# Autodesk Inventor assembly: Złożenie
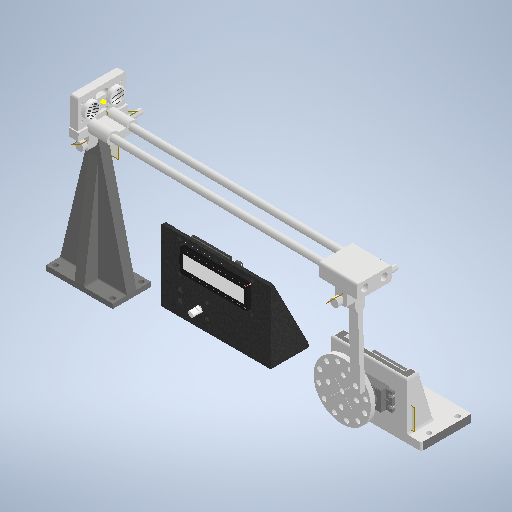
[picture p0: Inventor's stored thumbnail of the model, 512x512]
Saved by Autodesk Inventor 2025.2 (Build 292293000, 293)
## iProperties
Created: 2025-11-25
Part Number: Złożenie
Document SubType Name: Assembly
Designer: juras
Author: juras
## Documents named in this file (15)
- C:\Users\juras\Desktop\AiR SEMESTRY\AiR SEMESTR 5\SYSTEMY MIKROPROCESOROWE\LABORATORIUM\PROJEKT_KULKA_PID\KULKA_PID_KONSTRUKCJA\Złożenie.iam
- C:\Users\juras\Desktop\AiR SEMESTRY\AiR SEMESTR 5\SYSTEMY MIKROPROCESOROWE\LABORATORIUM\PROJEKT_KULKA_PID\KULKA_PID_KONSTRUKCJA\SG90_Arm_04_Custom\SG90_Arm_04_Custom\SG90_Arm_04_Custom.ipt
- C:\Users\juras\Desktop\AiR SEMESTRY\AiR SEMESTR 5\SYSTEMY MIKROPROCESOROWE\LABORATORIUM\PROJEKT_KULKA_PID\KULKA_PID_KONSTRUKCJA\DO_DRUKU_3D\Servo_przelozenie.ipt
- C:\Users\juras\Desktop\AiR SEMESTRY\AiR SEMESTR 5\SYSTEMY MIKROPROCESOROWE\LABORATORIUM\PROJEKT_KULKA_PID\KULKA_PID_KONSTRUKCJA\DO_DRUKU_3D\Czujnik_podstawa.ipt
- C:\Users\juras\Desktop\AiR SEMESTRY\AiR SEMESTR 5\SYSTEMY MIKROPROCESOROWE\LABORATORIUM\PROJEKT_KULKA_PID\KULKA_PID_KONSTRUKCJA\DO_DRUKU_3D\Toweript.ipt
- C:\Users\juras\Desktop\AiR SEMESTRY\AiR SEMESTR 5\SYSTEMY MIKROPROCESOROWE\LABORATORIUM\PROJEKT_KULKA_PID\KULKA_PID_KONSTRUKCJA\DO_DRUKU_3D\szpilka.ipt
- C:\Users\juras\Desktop\AiR SEMESTRY\AiR SEMESTR 5\SYSTEMY MIKROPROCESOROWE\LABORATORIUM\PROJEKT_KULKA_PID\KULKA_PID_KONSTRUKCJA\DO_DRUKU_3D\zaslepka.ipt
- C:\Users\juras\Desktop\AiR SEMESTRY\AiR SEMESTR 5\SYSTEMY MIKROPROCESOROWE\LABORATORIUM\PROJEKT_KULKA_PID\KULKA_PID_KONSTRUKCJA\HC-SR04 Sensor\HC-SR04 Sensor\HC-SR04 Sensor.ipt
- C:\Users\juras\Desktop\AiR SEMESTRY\AiR SEMESTR 5\SYSTEMY MIKROPROCESOROWE\LABORATORIUM\PROJEKT_KULKA_PID\KULKA_PID_KONSTRUKCJA\DO_DRUKU_3D\element_posredni.ipt
- C:\Users\juras\Desktop\AiR SEMESTRY\AiR SEMESTR 5\SYSTEMY MIKROPROCESOROWE\LABORATORIUM\PROJEKT_KULKA_PID\KULKA_PID_KONSTRUKCJA\DO_DRUKU_3D\sworzen.ipt
- C:\Users\juras\Desktop\AiR SEMESTRY\AiR SEMESTR 5\SYSTEMY MIKROPROCESOROWE\LABORATORIUM\PROJEKT_KULKA_PID\KULKA_PID_KONSTRUKCJA\DO_DRUKU_3D\LCD_podstawa.ipt
- C:\Users\juras\Desktop\AiR SEMESTRY\AiR SEMESTR 5\SYSTEMY MIKROPROCESOROWE\LABORATORIUM\PROJEKT_KULKA_PID\KULKA_PID_KONSTRUKCJA\1602A_I2C_LCD Module\1602A_I2C_LCD Module\1602A_I2C_LCD Module.ipt
- C:\Users\juras\Desktop\AiR SEMESTRY\AiR SEMESTR 5\SYSTEMY MIKROPROCESOROWE\LABORATORIUM\PROJEKT_KULKA_PID\KULKA_PID_KONSTRUKCJA\HW-040 Encoder module\HW-040 Encoder module\HW-040 Encoder module.iam
- C:\Users\juras\Desktop\AiR SEMESTRY\AiR SEMESTR 5\SYSTEMY MIKROPROCESOROWE\LABORATORIUM\PROJEKT_KULKA_PID\KULKA_PID_KONSTRUKCJA\mg996R_v2\mg996R_v2\mg996R_v2.ipt
- C:\Users\juras\Desktop\AiR SEMESTRY\AiR SEMESTR 5\SYSTEMY MIKROPROCESOROWE\LABORATORIUM\PROJEKT_KULKA_PID\KULKA_PID_KONSTRUKCJA\DO_DRUKU_3D\MG996R_PODSTAWA.ipt
## Components (16 placed, 14 different names)
1. SG90_Arm_04_Custom:1 — Zestawiające:45, Zestawiające:46, Zestawiające:81
2. Toweript:1 — Zestawiające:54, Zestawiające:55, Zestawiające:80, Zestawiające:82
3. zaslepka:1 — Zestawiające:47, Zestawiające:48, Zestawiające:60, Zestawiające:61, Zestawiające:62, Zestawiające:63
4. Servo_przelozenie:2 — Zestawiające:45, Zestawiające:46, Zestawiające:49, Zestawiające:50, Zestawiające:83
5. element_posredni:1 — Zestawiające:47, Zestawiające:48, Zestawiające:49, Zestawiające:50
6. Czujnik_podstawa:1 — Zestawiające:51, Zestawiające:52, Zestawiające:53, Zestawiające:54, Zestawiające:55, Zestawiające:56, Zestawiające:57, Zestawiające:58, Zestawiające:59, Zestawiające:64, Zestawiające:65
7. HC-SR04 Sensor:1 — Zestawiające:51, Zestawiające:52, Zestawiające:53
8. szpilka:1 — Zestawiające:56, Zestawiające:57, Zestawiające:61
9. szpilka:2 — Zestawiające:58, Zestawiające:59, Zestawiające:60
10. sworzen:1 — Zestawiające:62, Zestawiające:63
11. sworzen:2 — Zestawiające:64, Zestawiające:65
12. LCD_podstawa:1 — Zestawiające:70, Zestawiające:71, Zestawiające:72, Zestawiające:73, Zestawiające:78, Zestawiające:79, Zestawiające:80
13. 1602A_I2C_LCD Module:1 — Zestawiające:70, Zestawiające:71, Zestawiające:72
14. HW-040 Encoder module:1 [sub-assembly] — Zestawiające:73, Zestawiające:78
15. mg996R_v2:1 — Zestawiające:74, Zestawiające:75, Zestawiające:76, Zestawiające:77, Zestawiające:81, Zestawiające:83
16. MG996R_PODSTAWA:1 — Zestawiające:74, Zestawiające:75, Zestawiające:76, Zestawiające:77, Zestawiające:82
## Relationships (35: Mate 35)
- Zestawiające:45 [Mate]: SG90_Arm_04_Custom:1 ↔ Servo_przelozenie:2
- Zestawiające:46 [Mate]: SG90_Arm_04_Custom:1 ↔ Servo_przelozenie:2
- Zestawiające:47 [Mate]: zaslepka:1 ↔ element_posredni:1
- Zestawiające:48 [Mate]: zaslepka:1 ↔ element_posredni:1
- Zestawiające:49 [Mate]: Servo_przelozenie:2 ↔ element_posredni:1
- Zestawiające:50 [Mate]: Servo_przelozenie:2 ↔ element_posredni:1
- Zestawiające:51 [Mate]: Czujnik_podstawa:1 ↔ HC-SR04 Sensor:1
- Zestawiające:52 [Mate]: Czujnik_podstawa:1 ↔ HC-SR04 Sensor:1
- Zestawiające:53 [Mate]: Czujnik_podstawa:1 ↔ HC-SR04 Sensor:1
- Zestawiające:54 [Mate]: Toweript:1 ↔ Czujnik_podstawa:1
- Zestawiające:55 [Mate]: Toweript:1 ↔ Czujnik_podstawa:1
- Zestawiające:56 [Mate]: Czujnik_podstawa:1 ↔ szpilka:1
- Zestawiające:57 [Mate]: Czujnik_podstawa:1 ↔ szpilka:1
- Zestawiające:58 [Mate]: Czujnik_podstawa:1 ↔ szpilka:2
- Zestawiające:59 [Mate]: Czujnik_podstawa:1 ↔ szpilka:2
- Zestawiające:60 [Mate]: zaslepka:1 ↔ szpilka:2
- Zestawiające:61 [Mate]: zaslepka:1 ↔ szpilka:1
- Zestawiające:62 [Mate]: zaslepka:1 ↔ sworzen:1
- Zestawiające:63 [Mate] (2 mm): zaslepka:1 ↔ sworzen:1
- Zestawiające:64 [Mate]: Czujnik_podstawa:1 ↔ sworzen:2
- Zestawiające:65 [Mate]: Czujnik_podstawa:1 ↔ sworzen:2
- Zestawiające:70 [Mate]: LCD_podstawa:1 ↔ 1602A_I2C_LCD Module:1
- Zestawiające:71 [Mate]: LCD_podstawa:1 ↔ 1602A_I2C_LCD Module:1
- Zestawiające:72 [Mate]: LCD_podstawa:1 ↔ 1602A_I2C_LCD Module:1
- Zestawiające:73 [Mate]: LCD_podstawa:1 ↔ HW-040 Encoder module:1
- Zestawiające:74 [Mate]: mg996R_v2:1 ↔ MG996R_PODSTAWA:1
- Zestawiające:75 [Mate]: mg996R_v2:1 ↔ MG996R_PODSTAWA:1
- Zestawiające:76 [Mate]: mg996R_v2:1 ↔ MG996R_PODSTAWA:1
- Zestawiające:77 [Mate]: mg996R_v2:1 ↔ MG996R_PODSTAWA:1
- Zestawiające:78 [Mate]: LCD_podstawa:1 ↔ HW-040 Encoder module:1
- Zestawiające:79 [Mate] (-20 mm): LCD_podstawa:1
- Zestawiające:80 [Mate] (30 mm): Toweript:1 ↔ LCD_podstawa:1
- Zestawiające:81 [Mate]: SG90_Arm_04_Custom:1 ↔ mg996R_v2:1
- Zestawiające:82 [Mate]: Toweript:1 ↔ MG996R_PODSTAWA:1
- Zestawiające:83 [Mate]: Servo_przelozenie:2 ↔ mg996R_v2:1
